# Autodesk Inventor assembly: AssemblyTOT
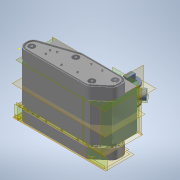
[picture p0: Inventor's stored thumbnail of the model, 180x180]
Saved by Autodesk Inventor 2021 (Build 250183000, 183)
## iProperties
Manager: PJ / DCS
Company: Emmaüs Bovenbouw Aalter
Created: 2020-11-25
Part Number: AssemblyTOT
Catalog Web Link: http://emmausbovenbouw.op-weg.be/
Vendor: Emmaüs Bovenbouw Aalter
Document SubType Name: Assembly
Designer: Antho
Engineer: Declercq St.
Authority: Declercq St.
Title: Algemene Projecttitel
Author: Antho
## Documents named in this file (5)
- C:\Users\Antho\Documents\Inventor\AssemblyTOT.iam
- C:\Users\Antho\Documents\Inventor\Assembly rupsbanden.iam
- C:\Users\Antho\Documents\Inventor\Assembly rupsband mirror_MIR1.iam
- C:\Users\Antho\Documents\Inventor\Behuizing.ipt
- C:\Users\Antho\Documents\Inventor\Scale Kannon.ipt
## Components (4 placed, 4 different names)
1. Assembly rupsbanden:1 [sub-assembly] — Mate:1, Flush:1, Flush:3, Flush:5
2. Mirror Rupsband assambly:1 [sub-assembly] — Mate:2, Flush:2, Flush:4
3. Behuizing:1 — Mate:1, Mate:2, Flush:1, Flush:2, Flush:3, Flush:4, Flush:7, Mate:4
4. Scale Kannon:1 — Mate:3, Mate:4, Flush:8
## Relationships (11: Flush 7, Mate 4)
- Mate:1: Assembly rupsbanden:1 ↔ Behuizing:1
- Mate:2: Mirror Rupsband assambly:1 ↔ Behuizing:1
- Flush:1: Assembly rupsbanden:1 ↔ Behuizing:1
- Flush:2: Mirror Rupsband assambly:1 ↔ Behuizing:1
- Flush:3: Assembly rupsbanden:1 ↔ Behuizing:1
- Flush:4: Mirror Rupsband assambly:1 ↔ Behuizing:1
- Flush:5 (75 mm): Assembly rupsbanden:1
- Flush:7 (75 mm): Behuizing:1
- Mate:3: Scale Kannon:1
- Mate:4: Behuizing:1 ↔ Scale Kannon:1
- Flush:8 (20 mm): Scale Kannon:1
